# Autodesk Inventor assembly: 付け根ロール_1
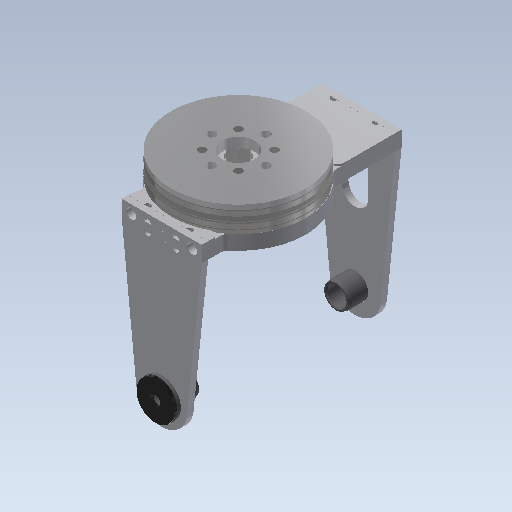
[picture p0: Inventor's stored thumbnail of the model, 512x512]
Saved by Autodesk Inventor 2020 (Build 240168000, 168)
## iProperties
Created: 2016-05-01
Part Number: 付け根ロール_1
Document SubType Name: Assembly
Designer: hiroaki
Mass: 101.489 g
Surface Area: 218.083 cm^2
Volume: 17.9148 cm^3
Density: 5.6651 g/cm^3
Author: hiroaki
## Documents named in this file (10)
- C:\Users\Masato\Desktop\最新版\OpenPlatform_ver3_0\下半身\付け根ロール\付け根ロール_1.iam
- C:\Users\Masato\Desktop\最新版\OpenPlatform_ver3_0\下半身\付け根ロール\付け根ロール_メインフレーム_1_1.ipt
- C:\Users\Masato\Desktop\最新版\OpenPlatform_ver3_0\Ready_Made\BA2542\BA2542.ipt
- C:\Users\Masato\Desktop\最新版\OpenPlatform_ver3_0\下半身\付け根ロール\付け根ロール_サブフレーム_1_4.ipt
- C:\Users\Masato\Desktop\最新版\OpenPlatform_ver3_0\Ready_Made\BA2542\BA2542_Washer.ipt
- C:\Users\Masato\Desktop\最新版\OpenPlatform_ver3_0\Ready_Made\MSU-306-03.ipt
- C:\Users\Masato\Desktop\最新版\OpenPlatform_ver3_0\下半身\付け根ロール\付け根ロール_サブフレーム_6_5.ipt
- C:\Users\Masato\Desktop\最新版\OpenPlatform_ver3_0\下半身\付け根ロール\付け根ロール_サブフレーム_6_6.ipt
- C:\Users\Masato\Desktop\最新版\OpenPlatform_ver3_0\Ready_Made\UUW-0312-10BH.ipt
- C:\Users\Masato\Desktop\最新版\OpenPlatform_ver3_0\Ready_Made\80F-0608.ipt
## Components (15 placed, 9 different names)
1. 付け根ロール_メインフレーム_1_1:1 — 挿入:29, 挿入:31, 挿入:32, 挿入:33, 挿入:34, 挿入:38, 挿入:39, 挿入:40, 挿入:41
2. BA2542:1 — 挿入:30
3. BA2542:2 — 挿入:24
4. 付け根ロール_サブフレーム_1_4:1 — 挿入:24, 挿入:35, 挿入:36, 挿入:37
5. BA2542_Washer:1 — 挿入:29, 挿入:30
6. MSU-306-03:1 — 挿入:31, 挿入:35
7. MSU-306-03:2 — 挿入:32, 挿入:36
8. MSU-306-03:3 — 挿入:33
9. MSU-306-03:4 — 挿入:34, 挿入:37
10. 付け根ロール_サブフレーム_6_5:1 — 挿入:40, 挿入:41, 挿入:48
11. 付け根ロール_サブフレーム_6_6:1 — 挿入:38, 挿入:39, 挿入:46
12. 80F-0608:1 — 挿入:46, 挿入:47
13. UUW-0312-10BH:3 — 挿入:47
14. 80F-0608:2 — 挿入:48, 挿入:49
15. UUW-0312-10BH:4 — 挿入:49
## Relationships (18: Insert 18)
- 挿入:24 [Insert]: BA2542:2 ↔ 付け根ロール_サブフレーム_1_4:1
- 挿入:29 [Insert]: 付け根ロール_メインフレーム_1_1:1 ↔ BA2542_Washer:1
- 挿入:30 [Insert]: BA2542:1 ↔ BA2542_Washer:1
- 挿入:31 [Insert]: 付け根ロール_メインフレーム_1_1:1 ↔ MSU-306-03:1
- 挿入:32 [Insert]: 付け根ロール_メインフレーム_1_1:1 ↔ MSU-306-03:2
- 挿入:33 [Insert]: 付け根ロール_メインフレーム_1_1:1 ↔ MSU-306-03:3
- 挿入:34 [Insert]: 付け根ロール_メインフレーム_1_1:1 ↔ MSU-306-03:4
- 挿入:35 [Insert]: 付け根ロール_サブフレーム_1_4:1 ↔ MSU-306-03:1
- 挿入:36 [Insert]: 付け根ロール_サブフレーム_1_4:1 ↔ MSU-306-03:2
- 挿入:37 [Insert]: 付け根ロール_サブフレーム_1_4:1 ↔ MSU-306-03:4
- 挿入:38 [Insert]: 付け根ロール_メインフレーム_1_1:1 ↔ 付け根ロール_サブフレーム_6_6:1
- 挿入:39 [Insert]: 付け根ロール_メインフレーム_1_1:1 ↔ 付け根ロール_サブフレーム_6_6:1
- 挿入:40 [Insert]: 付け根ロール_メインフレーム_1_1:1 ↔ 付け根ロール_サブフレーム_6_5:1
- 挿入:41 [Insert]: 付け根ロール_メインフレーム_1_1:1 ↔ 付け根ロール_サブフレーム_6_5:1
- 挿入:46 [Insert]: 付け根ロール_サブフレーム_6_6:1 ↔ 80F-0608:1
- 挿入:47 [Insert]: 80F-0608:1 ↔ UUW-0312-10BH:3
- 挿入:48 [Insert]: 付け根ロール_サブフレーム_6_5:1 ↔ 80F-0608:2
- 挿入:49 [Insert]: 80F-0608:2 ↔ UUW-0312-10BH:4
